# Autodesk Inventor assembly: PruebaIntegracion
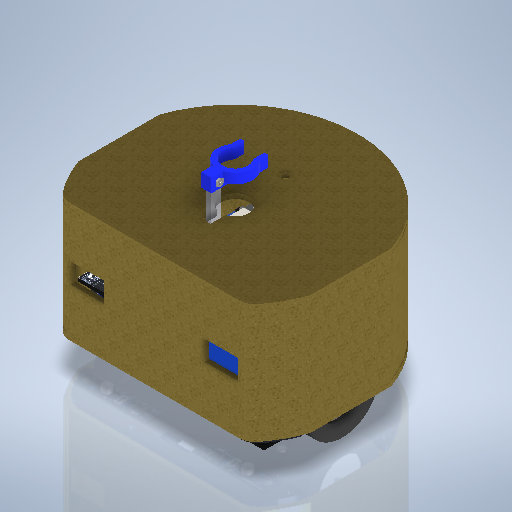
[picture p0: Inventor's stored thumbnail of the model, 512x512]
Saved by Autodesk Inventor 2025.2 (Build 292293000, 293)
## iProperties
Created: 2025-04-23
Part Number: PruebaIntegracion
Document SubType Name: Assembly
Designer: cdavi
Author: cdavi
## Documents named in this file (34)
- D:\Documentos\GIRoM\Atta-Bot-STEM\Chasis\Rediseño_Diego&Carlos\PruebaIntegracion.iam
- D:\Documentos\GIRoM\Atta-Bot-STEM\Chasis\Rediseño_Diego&Carlos\base_chasis_v5\base_chasis_v4-dimsAjustadas.ipt
- D:\Documentos\GIRoM\Atta-Bot-STEM\Chasis\Rediseño_Diego&Carlos\base_chasis_v5.ipt
- D:\Documentos\GIRoM\Atta-Bot-STEM\Chasis\Rediseño_Diego&Carlos\base_nivel2.ipt
- D:\Documentos\GIRoM\Atta-Bot-STEM\Chasis\Rediseño_Diego&Carlos\spacers\hexagonal_spacer_MF_M3_H20_HEX5.5_FTD6_MTL6.ipt
- D:\Documentos\GIRoM\Atta-Bot-STEM\Chasis\Rediseño_Diego&Carlos\spacers\hexagonal_spacer_MF_M3_H06_HEX5.5_FTD3_MTL6.ipt
- D:\Documentos\GIRoM\Atta-Bot-STEM\Chasis\Rediseño_Diego&Carlos\base_powerboost.ipt
- D:\Documentos\GIRoM\Atta-Bot-STEM\Chasis\Rediseño_Diego&Carlos\ideaboard.ipt
- D:\Documentos\GIRoM\Atta-Bot-STEM\Chasis\Rediseño_Diego&Carlos\sensorFrontal.ipt
- D:\Documentos\GIRoM\Atta-Bot-STEM\Chasis\Rediseño_Diego&Carlos\sensorInferior.ipt
- D:\Documentos\GIRoM\Atta-Bot-STEM\Chasis\Rediseño_Diego&Carlos\powerboost.ipt
- D:\Documentos\GIRoM\Atta-Bot-STEM\Chasis\Rediseño_Diego&Carlos\bateria.ipt
- D:\Documentos\GIRoM\Atta-Bot-STEM\Chasis\Rediseño_Diego&Carlos\soporteMotor.ipt
- D:\Documentos\GIRoM\Atta-Bot-STEM\Chasis\Rediseño_Diego&Carlos\motor.ipt
- D:\Documentos\GIRoM\Atta-Bot-STEM\Chasis\Rediseño_Diego&Carlos\llanta.ipt
- D:\Documentos\GIRoM\Atta-Bot-STEM\Chasis\Rediseño_Diego&Carlos\ball_caster.ipt
- D:\Documentos\GIRoM\Atta-Bot-STEM\Chasis\Rediseño_Diego&Carlos\switch.ipt
- D:\Documentos\GIRoM\Atta-Bot-STEM\Chasis\Rediseño_Diego&Carlos\Tower Pro MG90S Micro servo.ipt
- D:\Documentos\GIRoM\Atta-Bot-STEM\Chasis\Rediseño_Diego&Carlos\EngraneMod_v2.ipt
- D:\Documentos\GIRoM\Atta-Bot-STEM\Chasis\Rediseño_Diego&Carlos\sujetador_cremallera.ipt
- D:\Documentos\GIRoM\Atta-Bot-STEM\Chasis\Rediseño_Diego&Carlos\cremallera_v2\cremallera-01.ipt
- D:\Documentos\GIRoM\Atta-Bot-STEM\Chasis\Rediseño_Diego&Carlos\cremallera_v2.ipt
- D:\Documentos\GIRoM\Atta-Bot-STEM\Chasis\Rediseño_Diego&Carlos\sujetador_marcador_v2.ipt
- D:\Documentos\GIRoM\Atta-Bot-STEM\Chasis\Rediseño_Diego&Carlos\SoporteServo.ipt
- D:\Documentos\GIRoM\Atta-Bot-STEM\Chasis\Rediseño_Diego&Carlos\spacers\hexagonal_spacer_MF_M3_H08_HEX5_FTD4_MTL8.ipt
- D:\Documentos\GIRoM\Atta-Bot-STEM\Chasis\Rediseño_Diego&Carlos\Content Center Files\en-US\ISO 4032(2)\ISO 4032 - M3 - ISO.ipt
- D:\Documentos\GIRoM\Atta-Bot-STEM\Chasis\Rediseño_Diego&Carlos\Content Center Files\en-US\ISO 7045  Z\ISO 7045 - M3 x 6_ - 4.8 - Z - ISO.ipt
- D:\Documentos\GIRoM\Atta-Bot-STEM\Chasis\Rediseño_Diego&Carlos\Content Center Files\en-US\ISO 4762(2)\ISO 4762 - M3 x 12ISO.ipt
- D:\Documentos\GIRoM\Atta-Bot-STEM\Chasis\Rediseño_Diego&Carlos\Content Center Files\en-US\ISO 4032(2)\ISO 4032 - M2 - ISO.ipt
- D:\Documentos\GIRoM\Atta-Bot-STEM\Chasis\Rediseño_Diego&Carlos\Content Center Files\en-US\ISO 4762(2)\ISO 4762 - M2 x 8ISO.ipt
- D:\Documentos\GIRoM\Atta-Bot-STEM\Chasis\Rediseño_Diego&Carlos\Content Center Files\en-US\ISO 4762(2)\ISO 4762 - M2 x 12ISO.ipt
- D:\Documentos\GIRoM\Atta-Bot-STEM\Chasis\Rediseño_Diego&Carlos\Content Center Files\en-US\ISO 7045  Z\ISO 7045 - M1,6 x 6_ - 4.8 - Z - ISO.ipt
- D:\Documentos\GIRoM\Atta-Bot-STEM\Chasis\Rediseño_Diego&Carlos\Content Center Files\en-US\ISO 4762(2)\ISO 4762 - M3 x 8ISO.ipt
- D:\Documentos\GIRoM\Diseño mecánico\carcasa.ipt
## Components (106 placed, 31 different names)
1. carcasa:1 — Mate:217, Mate:218, Mate:219
2. hexagonal_spacer_MF_M3_H20_HEX5.5_FTD6_MTL6:1 — Mate:3, Mate:4, Mate:210, Mate:214
3. hexagonal_spacer_MF_M3_H20_HEX5.5_FTD6_MTL6:2 — Mate:5, Mate:6, Mate:211, Mate:212, Mate:216
4. hexagonal_spacer_MF_M3_H20_HEX5.5_FTD6_MTL6:3 — Mate:7, Mate:8, Mate:215
5. hexagonal_spacer_MF_M3_H20_HEX5.5_FTD6_MTL6:4 — Mate:9, Mate:10, Mate:213
6. hexagonal_spacer_MF_M3_H08_HEX5_FTD4_MTL8:2
7. hexagonal_spacer_MF_M3_H08_HEX5_FTD4_MTL8:1
8. hexagonal_spacer_MF_M3_H08_HEX5_FTD4_MTL8:3
9. hexagonal_spacer_MF_M3_H08_HEX5_FTD4_MTL8:4
10. hexagonal_spacer_MF_M3_H06_HEX5.5_FTD3_MTL6:2 — Mate:44, Mate:45
11. hexagonal_spacer_MF_M3_H06_HEX5.5_FTD3_MTL6:3 — Mate:48, Mate:49
12. hexagonal_spacer_MF_M3_H06_HEX5.5_FTD3_MTL6:1 — Mate:42, Mate:43, Mate:50, Mate:51
13. hexagonal_spacer_MF_M3_H06_HEX5.5_FTD3_MTL6:4 — Mate:46, Mate:47, Mate:52
14. hexagonal_spacer_MF_M3_H06_HEX5.5_FTD3_MTL6:5 — Mate:53, Mate:54, Mate:68, Mate:69, Mate:70
15. hexagonal_spacer_MF_M3_H06_HEX5.5_FTD3_MTL6:6 — Mate:55, Mate:56, Mate:66, Mate:67, Mate:73
16. ISO 4032 M3:37 — Mate:199, Mate:83
17. ISO 4032 M3:38 — Mate:201, Mate:85
18. ISO 7045 Z M3 x 6 - 4.8 - Z:25 — Insert:14
19. ISO 7045 Z M3 x 6 - 4.8 - Z:26 — Insert:15
20. ISO 4032 M3:39 — Insert:16
21. ISO 4032 M3:40 — Insert:17
22. ISO 4032 M3:41 — Insert:18
23. ISO 4032 M3:42 — Insert:19
24. ISO 4032 M3:43 — Insert:5
25. ISO 4032 M3:44 — Insert:6
26. ISO 4032 M3:45 — Insert:7
27. ISO 4032 M3:46 — Insert:8
28. ISO 7045 Z M3 x 6 - 4.8 - Z:27 — Insert:9
29. ISO 7045 Z M3 x 6 - 4.8 - Z:28 — Insert:10
30. ISO 4762 M3 x 12:5 — Insert:114
31. ISO 4762 M3 x 12:6 — Mate:115, Mate:116
32. ISO 7045 Z M3 x 6 - 4.8 - Z:29 — Mate:89, Mate:90
33. ISO 7045 Z M3 x 6 - 4.8 - Z:30 — Mate:91, Mate:92
34. ISO 7045 Z M3 x 6 - 4.8 - Z:31 — Mate:93, Mate:94
35. ISO 7045 Z M3 x 6 - 4.8 - Z:32 — Mate:95, Mate:96
36. ISO 4032 M3:47 — Mate:58, Mate:215
37. ISO 4032 M3:48 — Mate:60, Mate:216
38. ISO 4032 M3:49 — Mate:63, Mate:214
39. ISO 4032 M3:50 — Mate:64, Mate:213
40. ISO 4032 M3:51 — Mate:70, Mate:71
41. ISO 4032 M3:52 — Mate:72, Mate:73
42. ISO 7045 Z M3 x 6 - 4.8 - Z:33 — Mate:74, Mate:75
43. ISO 7045 Z M3 x 6 - 4.8 - Z:34 — Mate:76, Mate:77
44. ISO 7045 Z M3 x 6 - 4.8 - Z:35 — Mate:78, Mate:79
45. ISO 7045 Z M3 x 6 - 4.8 - Z:36 — Mate:80, Mate:81
46. ISO 4032 M2:18 — Mate:189, Mate:190
47. ISO 4032 M2:19 — Mate:191, Mate:192
48. ISO 4032 M2:20 — Mate:194, Mate:197
49. ISO 4032 M2:21 — Mate:196
50. ISO 4762 M2 x 8:19 — Mate:148, Mate:149, Mate:154
51. ISO 4762 M2 x 8:20 — Mate:150, Mate:151, Mate:152
52. ISO 4032 M2:22 — Mate:152, Mate:153
53. ISO 4032 M2:23 — Mate:154, Mate:155
54. ISO 4032 M2:24 — Mate:160, Mate:161
55. ISO 4032 M2:25 — Mate:162, Mate:163
56. ISO 4032 M2:26 — Mate:164, Mate:165
57. ISO 4032 M2:27 — Mate:166, Mate:167
58. ISO 4762 M2 x 8:21 — Mate:160
59. ISO 4762 M2 x 8:22 — Mate:162
60. ISO 4762 M2 x 8:23 — Mate:166
61. ISO 4762 M2 x 8:24 — Mate:164
62. ISO 4762 M2 x 8:25 — Mate:97, Mate:98, Mate:110, Mate:191
63. ISO 4762 M2 x 8:26 — Mate:99, Mate:100, Mate:112, Mate:189
64. ISO 4762 M2 x 12:7
65. ISO 4762 M2 x 12:8
66. ISO 4032 M2:28 — Mate:106
67. ISO 4032 M2:29 — Mate:107
68. ISO 4032 M2:30 — Mate:109, Mate:110
69. ISO 4032 M2:31 — Mate:111, Mate:112
70. ISO 7045 Z M1,6 x 6 - 4.8 - Z:4 — Mate:156, Mate:157
71. ISO 7045 Z M1,6 x 6 - 4.8 - Z:5 — Mate:158, Mate:159
72. bateria:1 — Mate:119, Mate:120
73. soporteMotor:1 — Mate:117, Mate:118, Angle:8, Mate:124, Tangent:2
74. soporteMotor:2 — Mate:119, Mate:122, Tangent:1, Mate:181, Angle:12, Mate:182
75. motor:1 — Mate:122, Tangent:1, Mate:123, Mate:126, Flush:5, Mate:127
76. motor:2 — Mate:124, Tangent:2, Mate:125, Mate:128, Mate:129, Flush:6
77. llanta:1 — Mate:126, Flush:5, Mate:127
78. llanta:2 — Mate:128, Mate:129, Flush:6
79. ball_caster:1 — Tangent:3, Tangent:7, Mate:130, Mate:156, Mate:158
80. switch:1 — Mate:131, Mate:132, Mate:133, Mate:148, Mate:149, Mate:150, Mate:151
81. sensorInferior:2 — Angle:7, Mate:85, Insert:114, Mate:82
82. sensorInferior:1 — Angle:6, Mate:83, Mate:115, Mate:116, Mate:84
83. powerboost:1 — Mate:86, Mate:87, Mate:88, Mate:97, Mate:98, Mate:99, Mate:100, Mate:197
84. base_chasis_v4-dimsAjustadas:1 — Mate:1, Flush:8, Flush:4, Mate:3, Mate:4, Mate:5, Mate:6, Mate:7, Mate:8, Mate:9, Mate:10, Mate:82, Angle:6, Mate:84, Angle:7, Mate:117, Mate:118, Angle:8, Mate:120, Mate:123, Mate:125, Tangent:3, Tangent:7, Mate:130, Mate:131, Mate:132, Mate:133, Mate:153, Mate:155, Mate:157, Mate:159, Mate:161, Mate:163, Mate:165, Mate:167, Insert:5, Insert:6, Insert:7, Insert:8, Insert:9, Insert:10, Mate:181, Angle:12, Mate:182, Mate:199, Mate:201, Mate:217, Mate:218, Mate:219
85. base_powerboost:1 — Mate:86, Mate:87, Mate:88, Mate:89, Mate:90, Mate:91, Mate:92, Mate:93, Mate:94, Mate:95, Mate:96, Mate:106, Mate:107, Mate:109, Mate:111, Mate:190, Mate:192, Mate:194, Mate:196
86. SoporteServo:2 — Mate:186, Mate:187, Mate:188, Mate:209
87. base_nivel2:1 — Mate:42, Mate:43, Mate:44, Mate:45, Mate:46, Mate:47, Mate:48, Mate:49, Mate:53, Mate:54, Mate:55, Mate:56, Mate:58, Mate:60, Mate:63, Mate:64, Angle:4, Angle:5, Angle:9, Insert:14, Insert:15, Insert:16, Insert:17, Insert:18, Insert:19, Flush:7, Mate:186, Mate:187, Mate:210, Mate:211, Mate:212
88. SoporteServo:1 — Mate:208
89. ideaboard:1 — Mate:50, Mate:51, Mate:52, Mate:74, Mate:75, Mate:76, Mate:77, Mate:78, Mate:79, Mate:80, Mate:81
90. sensorFrontal:1 — Mate:66, Mate:67, Angle:4, Mate:72
91. sensorFrontal:2 — Mate:68, Mate:69, Angle:5, Mate:71
92. ISO 4032 M2:32 — Mate:208
93. ISO 4032 M2:33 — Mate:209
94. ISO 4762 M2 x 12:9
95. ISO 4762 M3 x 8:3 — Mate:202, Mate:203, Mate:206
96. ISO 4762 M3 x 8:4 — Mate:204, Mate:205, Mate:207
97. ISO 4032 M3:53 — Mate:169, Mate:206
98. ISO 4032 M3:54 — Mate:171, Mate:207
99. ISO 4762 M2 x 12:10
100. Tower Pro MG90S Micro servo:1 — Angle:9, Mate:136, Mate:138, Angle:10, Mate:143, Flush:7, Mate:188
101. EngraneMod_v2:1 — Mate:136, Mate:139, Mate:143
102. sujetador_cremallera:1 — Mate:138, Angle:10, Mate:139, Tangent:5, Tangent:6, Mate:140, Mate:203, Mate:205, Mate:169, Mate:171
103. cremallera-01:1 — Tangent:5, Tangent:6, Mate:140, Mate:141, Angle:11, Mate:142, Mate:202, Mate:204
104. sujetador_marcador_v2:1 — Mate:141, Angle:11, Mate:142, Mate:144, Mate:145, Mate:147
105. ISO 4762 M2 x 8:27 — Mate:144, Mate:145, Mate:146
106. ISO 4032 M2:34 — Mate:146, Mate:147
## Relationships (218: Mate 180, Insert 18, Angle 9, Tangent 6, Flush 5)
- Mate:1: base_chasis_v4-dimsAjustadas:1
- Flush:8: base_chasis_v4-dimsAjustadas:1
- Flush:4: base_chasis_v4-dimsAjustadas:1
- Mate:3: hexagonal_spacer_MF_M3_H20_HEX5.5_FTD6_MTL6:1 ↔ base_chasis_v4-dimsAjustadas:1
- Mate:4: hexagonal_spacer_MF_M3_H20_HEX5.5_FTD6_MTL6:1 ↔ base_chasis_v4-dimsAjustadas:1
- Mate:5: hexagonal_spacer_MF_M3_H20_HEX5.5_FTD6_MTL6:2 ↔ base_chasis_v4-dimsAjustadas:1
- Mate:6: hexagonal_spacer_MF_M3_H20_HEX5.5_FTD6_MTL6:2 ↔ base_chasis_v4-dimsAjustadas:1
- Mate:7: hexagonal_spacer_MF_M3_H20_HEX5.5_FTD6_MTL6:3 ↔ base_chasis_v4-dimsAjustadas:1
- Mate:8: hexagonal_spacer_MF_M3_H20_HEX5.5_FTD6_MTL6:3 ↔ base_chasis_v4-dimsAjustadas:1
- Mate:9: hexagonal_spacer_MF_M3_H20_HEX5.5_FTD6_MTL6:4 ↔ base_chasis_v4-dimsAjustadas:1
- Mate:10: hexagonal_spacer_MF_M3_H20_HEX5.5_FTD6_MTL6:4 ↔ base_chasis_v4-dimsAjustadas:1
- [Mate]: hexagonal_spacer_MF_M3_H08_HEX5_FTD4_MTL8:2 ↔ base_chasis_v4-dimsAjustadas:1
- [Mate]: hexagonal_spacer_MF_M3_H08_HEX5_FTD4_MTL8:2 ↔ base_chasis_v4-dimsAjustadas:1
- [Mate]: hexagonal_spacer_MF_M3_H08_HEX5_FTD4_MTL8:1 ↔ base_chasis_v4-dimsAjustadas:1
- [Mate]: hexagonal_spacer_MF_M3_H08_HEX5_FTD4_MTL8:1 ↔ base_chasis_v4-dimsAjustadas:1
- [Mate]: hexagonal_spacer_MF_M3_H08_HEX5_FTD4_MTL8:3 ↔ base_chasis_v4-dimsAjustadas:1
- [Mate]: hexagonal_spacer_MF_M3_H08_HEX5_FTD4_MTL8:3 ↔ base_chasis_v4-dimsAjustadas:1
- [Mate]: hexagonal_spacer_MF_M3_H08_HEX5_FTD4_MTL8:4 ↔ base_chasis_v4-dimsAjustadas:1
- [Mate]: hexagonal_spacer_MF_M3_H08_HEX5_FTD4_MTL8:4 ↔ base_chasis_v4-dimsAjustadas:1
- [Mate]: hexagonal_spacer_MF_M3_H08_HEX5_FTD4_MTL8:3 ↔ base_powerboost:1
- [Mate]: hexagonal_spacer_MF_M3_H08_HEX5_FTD4_MTL8:2 ↔ base_powerboost:1
- [Mate]: hexagonal_spacer_MF_M3_H08_HEX5_FTD4_MTL8:2 ↔ base_powerboost:1
- [Mate]: base_nivel2:1 ↔ SoporteServo:1
- [Mate]: base_nivel2:1 ↔ SoporteServo:1
- [Mate]: base_nivel2:1 ↔ SoporteServo:1
- Mate:42: hexagonal_spacer_MF_M3_H06_HEX5.5_FTD3_MTL6:1 ↔ base_nivel2:1
- Mate:43: hexagonal_spacer_MF_M3_H06_HEX5.5_FTD3_MTL6:1 ↔ base_nivel2:1
- Mate:44: hexagonal_spacer_MF_M3_H06_HEX5.5_FTD3_MTL6:2 ↔ base_nivel2:1
- Mate:45: hexagonal_spacer_MF_M3_H06_HEX5.5_FTD3_MTL6:2 ↔ base_nivel2:1
- Mate:46: hexagonal_spacer_MF_M3_H06_HEX5.5_FTD3_MTL6:4 ↔ base_nivel2:1
- Mate:47: hexagonal_spacer_MF_M3_H06_HEX5.5_FTD3_MTL6:4 ↔ base_nivel2:1
- Mate:48: hexagonal_spacer_MF_M3_H06_HEX5.5_FTD3_MTL6:3 ↔ base_nivel2:1
- Mate:49: hexagonal_spacer_MF_M3_H06_HEX5.5_FTD3_MTL6:3 ↔ base_nivel2:1
- Mate:50: hexagonal_spacer_MF_M3_H06_HEX5.5_FTD3_MTL6:1 ↔ ideaboard:1
- Mate:51: hexagonal_spacer_MF_M3_H06_HEX5.5_FTD3_MTL6:1 ↔ ideaboard:1
- Mate:52: hexagonal_spacer_MF_M3_H06_HEX5.5_FTD3_MTL6:4 ↔ ideaboard:1
- Mate:53: hexagonal_spacer_MF_M3_H06_HEX5.5_FTD3_MTL6:5 ↔ base_nivel2:1
- Mate:54: hexagonal_spacer_MF_M3_H06_HEX5.5_FTD3_MTL6:5 ↔ base_nivel2:1
- Mate:55: hexagonal_spacer_MF_M3_H06_HEX5.5_FTD3_MTL6:6 ↔ base_nivel2:1
- Mate:56: hexagonal_spacer_MF_M3_H06_HEX5.5_FTD3_MTL6:6 ↔ base_nivel2:1
- Mate:58: ISO 4032 M3:47 ↔ base_nivel2:1
- Mate:60: ISO 4032 M3:48 ↔ base_nivel2:1
- Mate:63: ISO 4032 M3:49 ↔ base_nivel2:1
- Mate:64: ISO 4032 M3:50 ↔ base_nivel2:1
- Mate:66: hexagonal_spacer_MF_M3_H06_HEX5.5_FTD3_MTL6:6 ↔ sensorFrontal:1
- Mate:67: hexagonal_spacer_MF_M3_H06_HEX5.5_FTD3_MTL6:6 ↔ sensorFrontal:1
- Angle:4 (180 deg): base_nivel2:1 ↔ sensorFrontal:1
- Mate:68: hexagonal_spacer_MF_M3_H06_HEX5.5_FTD3_MTL6:5 ↔ sensorFrontal:2
- Mate:69: hexagonal_spacer_MF_M3_H06_HEX5.5_FTD3_MTL6:5 ↔ sensorFrontal:2
- Angle:5 (0 deg): base_nivel2:1 ↔ sensorFrontal:2
- Mate:70: hexagonal_spacer_MF_M3_H06_HEX5.5_FTD3_MTL6:5 ↔ ISO 4032 M3:51
- Mate:71: ISO 4032 M3:51 ↔ sensorFrontal:2
- Mate:72: ISO 4032 M3:52 ↔ sensorFrontal:1
- Mate:73: hexagonal_spacer_MF_M3_H06_HEX5.5_FTD3_MTL6:6 ↔ ISO 4032 M3:52
- Mate:74: ISO 7045 Z M3 x 6 - 4.8 - Z:33 ↔ ideaboard:1
- Mate:75: ISO 7045 Z M3 x 6 - 4.8 - Z:33 ↔ ideaboard:1
- Mate:76: ISO 7045 Z M3 x 6 - 4.8 - Z:34 ↔ ideaboard:1
- Mate:77: ISO 7045 Z M3 x 6 - 4.8 - Z:34 ↔ ideaboard:1
- Mate:78: ISO 7045 Z M3 x 6 - 4.8 - Z:35 ↔ ideaboard:1
- Mate:79: ISO 7045 Z M3 x 6 - 4.8 - Z:35 ↔ ideaboard:1
- Mate:80: ISO 7045 Z M3 x 6 - 4.8 - Z:36 ↔ ideaboard:1
- Mate:81: ISO 7045 Z M3 x 6 - 4.8 - Z:36 ↔ ideaboard:1
- Mate:82: sensorInferior:2 ↔ base_chasis_v4-dimsAjustadas:1
- Angle:6 (0 deg): sensorInferior:1 ↔ base_chasis_v4-dimsAjustadas:1
- Mate:83: ISO 4032 M3:37 ↔ sensorInferior:1
- Mate:84: sensorInferior:1 ↔ base_chasis_v4-dimsAjustadas:1
- Angle:7 (0 deg): sensorInferior:2 ↔ base_chasis_v4-dimsAjustadas:1
- Mate:85: ISO 4032 M3:38 ↔ sensorInferior:2
- Mate:86: powerboost:1 ↔ base_powerboost:1
- Mate:87: powerboost:1 ↔ base_powerboost:1
- Mate:88 (1 mm): powerboost:1 ↔ base_powerboost:1
- Mate:89: ISO 7045 Z M3 x 6 - 4.8 - Z:29 ↔ base_powerboost:1
- Mate:90: ISO 7045 Z M3 x 6 - 4.8 - Z:29 ↔ base_powerboost:1
- Mate:91: ISO 7045 Z M3 x 6 - 4.8 - Z:30 ↔ base_powerboost:1
- Mate:92: ISO 7045 Z M3 x 6 - 4.8 - Z:30 ↔ base_powerboost:1
- Mate:93: ISO 7045 Z M3 x 6 - 4.8 - Z:31 ↔ base_powerboost:1
- Mate:94: ISO 7045 Z M3 x 6 - 4.8 - Z:31 ↔ base_powerboost:1
- Mate:95: ISO 7045 Z M3 x 6 - 4.8 - Z:32 ↔ base_powerboost:1
- Mate:96: ISO 7045 Z M3 x 6 - 4.8 - Z:32 ↔ base_powerboost:1
- Mate:97: ISO 4762 M2 x 8:25 ↔ powerboost:1
- Mate:98: ISO 4762 M2 x 8:25 ↔ powerboost:1
- Mate:99: ISO 4762 M2 x 8:26 ↔ powerboost:1
- Mate:100: ISO 4762 M2 x 8:26 ↔ powerboost:1
- [Mate]: ISO 4762 M2 x 12:7 ↔ powerboost:1
- [Mate]: ISO 4762 M2 x 12:7 ↔ powerboost:1
- [Mate]: ISO 4762 M2 x 12:8 ↔ powerboost:1
- [Mate]: ISO 4762 M2 x 12:8 ↔ powerboost:1
- [Mate]: ISO 4762 M2 x 12:7 ↔ ISO 4032 M2:28
- Mate:106: ISO 4032 M2:28 ↔ base_powerboost:1
- Mate:107: ISO 4032 M2:29 ↔ base_powerboost:1
- [Mate]: ISO 4762 M2 x 12:8 ↔ ISO 4032 M2:29
- Mate:109: ISO 4032 M2:30 ↔ base_powerboost:1
- Mate:110: ISO 4762 M2 x 8:25 ↔ ISO 4032 M2:30
- Mate:111: ISO 4032 M2:31 ↔ base_powerboost:1
- Mate:112: ISO 4762 M2 x 8:26 ↔ ISO 4032 M2:31
- Insert:114: ISO 4762 M3 x 12:5 ↔ sensorInferior:2
- Mate:115: ISO 4762 M3 x 12:6 ↔ sensorInferior:1
- Mate:116: ISO 4762 M3 x 12:6 ↔ sensorInferior:1
- Mate:117: soporteMotor:1 ↔ base_chasis_v4-dimsAjustadas:1
- Mate:118: soporteMotor:1 ↔ base_chasis_v4-dimsAjustadas:1
- Angle:8 (0 deg): soporteMotor:1 ↔ base_chasis_v4-dimsAjustadas:1
- Mate:119: bateria:1 ↔ soporteMotor:2
- Mate:120: bateria:1 ↔ base_chasis_v4-dimsAjustadas:1
- [Mate] (1 mm): hexagonal_spacer_MF_M3_H08_HEX5_FTD4_MTL8:1 ↔ bateria:1
- Mate:122: soporteMotor:2 ↔ motor:1
- Tangent:1: soporteMotor:2 ↔ motor:1
- Mate:123: motor:1 ↔ base_chasis_v4-dimsAjustadas:1
- Mate:124: soporteMotor:1 ↔ motor:2
- Tangent:2: soporteMotor:1 ↔ motor:2
- Mate:125: motor:2 ↔ base_chasis_v4-dimsAjustadas:1
- Mate:126: motor:1 ↔ llanta:1
- Flush:5 (-3 mm): motor:1 ↔ llanta:1
- Mate:127: motor:1 ↔ llanta:1
- Mate:128: motor:2 ↔ llanta:2
- Mate:129: motor:2 ↔ llanta:2
- Flush:6 (-3 mm): motor:2 ↔ llanta:2
- Tangent:3: ball_caster:1 ↔ base_chasis_v4-dimsAjustadas:1
- Tangent:7: ball_caster:1 ↔ base_chasis_v4-dimsAjustadas:1
- Mate:130: ball_caster:1 ↔ base_chasis_v4-dimsAjustadas:1
- Mate:131: switch:1 ↔ base_chasis_v4-dimsAjustadas:1
- Mate:132: switch:1 ↔ base_chasis_v4-dimsAjustadas:1
- Mate:133 (0.2 mm): switch:1 ↔ base_chasis_v4-dimsAjustadas:1
- [Mate]: SoporteServo:1 ↔ Tower Pro MG90S Micro servo:1
- Angle:9 (180 deg): base_nivel2:1 ↔ Tower Pro MG90S Micro servo:1
- Mate:136: Tower Pro MG90S Micro servo:1 ↔ EngraneMod_v2:1
- Mate:138: Tower Pro MG90S Micro servo:1 ↔ sujetador_cremallera:1
- Angle:10 (0 deg): Tower Pro MG90S Micro servo:1 ↔ sujetador_cremallera:1
- Mate:139: EngraneMod_v2:1 ↔ sujetador_cremallera:1
- Tangent:5: sujetador_cremallera:1 ↔ cremallera-01:1
- Tangent:6: sujetador_cremallera:1 ↔ cremallera-01:1
- Mate:140: sujetador_cremallera:1 ↔ cremallera-01:1
- Mate:141: cremallera-01:1 ↔ sujetador_marcador_v2:1
- Angle:11 (0 deg): cremallera-01:1 ↔ sujetador_marcador_v2:1
- Mate:142: cremallera-01:1 ↔ sujetador_marcador_v2:1
- Mate:143: Tower Pro MG90S Micro servo:1 ↔ EngraneMod_v2:1
- Mate:144: sujetador_marcador_v2:1 ↔ ISO 4762 M2 x 8:27
- Mate:145: sujetador_marcador_v2:1 ↔ ISO 4762 M2 x 8:27
- Mate:146: ISO 4762 M2 x 8:27 ↔ ISO 4032 M2:34
- Mate:147: sujetador_marcador_v2:1 ↔ ISO 4032 M2:34
- Mate:148: ISO 4762 M2 x 8:19 ↔ switch:1
- Mate:149: ISO 4762 M2 x 8:19 ↔ switch:1
- Mate:150: ISO 4762 M2 x 8:20 ↔ switch:1
- Mate:151: ISO 4762 M2 x 8:20 ↔ switch:1
- Mate:152: ISO 4762 M2 x 8:20 ↔ ISO 4032 M2:22
- Mate:153: ISO 4032 M2:22 ↔ base_chasis_v4-dimsAjustadas:1
- Mate:154: ISO 4762 M2 x 8:19 ↔ ISO 4032 M2:23
- Mate:155: ISO 4032 M2:23 ↔ base_chasis_v4-dimsAjustadas:1
- Mate:156: ISO 7045 Z M1,6 x 6 - 4.8 - Z:4 ↔ ball_caster:1
- Mate:157: ISO 7045 Z M1,6 x 6 - 4.8 - Z:4 ↔ base_chasis_v4-dimsAjustadas:1
- Mate:158: ISO 7045 Z M1,6 x 6 - 4.8 - Z:5 ↔ ball_caster:1
- Mate:159: ISO 7045 Z M1,6 x 6 - 4.8 - Z:5 ↔ base_chasis_v4-dimsAjustadas:1
- [Insert]: ISO 4762 M2 x 8:21 ↔ soporteMotor:2
- [Insert]: ISO 4762 M2 x 8:22 ↔ soporteMotor:2
- [Insert]: ISO 4762 M2 x 8:23 ↔ soporteMotor:1
- [Insert]: ISO 4762 M2 x 8:24 ↔ soporteMotor:1
- Mate:160: ISO 4032 M2:24 ↔ ISO 4762 M2 x 8:21
- Mate:161: ISO 4032 M2:24 ↔ base_chasis_v4-dimsAjustadas:1
- Mate:162: ISO 4032 M2:25 ↔ ISO 4762 M2 x 8:22
- Mate:163: ISO 4032 M2:25 ↔ base_chasis_v4-dimsAjustadas:1
- Mate:164: ISO 4032 M2:26 ↔ ISO 4762 M2 x 8:24
- Mate:165: ISO 4032 M2:26 ↔ base_chasis_v4-dimsAjustadas:1
- Mate:166: ISO 4032 M2:27 ↔ ISO 4762 M2 x 8:23
- Mate:167: ISO 4032 M2:27 ↔ base_chasis_v4-dimsAjustadas:1
- Insert:5: ISO 4032 M3:43 ↔ base_chasis_v4-dimsAjustadas:1
- Insert:6: ISO 4032 M3:44 ↔ base_chasis_v4-dimsAjustadas:1
- Insert:7: ISO 4032 M3:45 ↔ base_chasis_v4-dimsAjustadas:1
- Insert:8: ISO 4032 M3:46 ↔ base_chasis_v4-dimsAjustadas:1
- Insert:9: ISO 7045 Z M3 x 6 - 4.8 - Z:27 ↔ base_chasis_v4-dimsAjustadas:1
- Insert:10: ISO 7045 Z M3 x 6 - 4.8 - Z:28 ↔ base_chasis_v4-dimsAjustadas:1
- Mate:169: ISO 4032 M3:53 ↔ sujetador_cremallera:1
- Mate:171: ISO 4032 M3:54 ↔ sujetador_cremallera:1
- [Mate]: ISO 4762 M2 x 12:10 ↔ Tower Pro MG90S Micro servo:1
- [Mate]: ISO 4762 M2 x 12:10 ↔ Tower Pro MG90S Micro servo:1
- [Insert]: ISO 4762 M2 x 12:9 ↔ Tower Pro MG90S Micro servo:1
- [Mate]: ISO 4032 M2:33 ↔ ISO 4762 M2 x 12:9
- [Mate]: ISO 4032 M2:32 ↔ ISO 4762 M2 x 12:10
- Insert:14: ISO 7045 Z M3 x 6 - 4.8 - Z:25 ↔ base_nivel2:1
- Insert:15: ISO 7045 Z M3 x 6 - 4.8 - Z:26 ↔ base_nivel2:1
- Insert:16: ISO 4032 M3:39 ↔ base_nivel2:1
- Insert:17: ISO 4032 M3:40 ↔ base_nivel2:1
- Insert:18: ISO 4032 M3:41 ↔ base_nivel2:1
- Insert:19: ISO 4032 M3:42 ↔ base_nivel2:1
- Flush:7: base_nivel2:1 ↔ Tower Pro MG90S Micro servo:1
- Mate:181: soporteMotor:2 ↔ base_chasis_v4-dimsAjustadas:1
- Angle:12 (0 deg): soporteMotor:2 ↔ base_chasis_v4-dimsAjustadas:1
- Mate:182: soporteMotor:2 ↔ base_chasis_v4-dimsAjustadas:1
- Mate:186: SoporteServo:2 ↔ base_nivel2:1
- Mate:187: SoporteServo:2 ↔ base_nivel2:1
- Mate:188: SoporteServo:2 ↔ Tower Pro MG90S Micro servo:1
- Mate:189: ISO 4032 M2:18 ↔ ISO 4762 M2 x 8:26
- Mate:190: ISO 4032 M2:18 ↔ base_powerboost:1
- Mate:191: ISO 4032 M2:19 ↔ ISO 4762 M2 x 8:25
- Mate:192: ISO 4032 M2:19 ↔ base_powerboost:1
- [Mate]: ISO 4032 M2:20 ↔ ISO 4762 M2 x 12:8
- Mate:194: ISO 4032 M2:20 ↔ base_powerboost:1
- [Mate]: ISO 4032 M2:21 ↔ ISO 4762 M2 x 12:7
- Mate:196: ISO 4032 M2:21 ↔ base_powerboost:1
- Mate:197: ISO 4032 M2:20 ↔ powerboost:1
- Mate:199: ISO 4032 M3:37 ↔ base_chasis_v4-dimsAjustadas:1
- Mate:201: ISO 4032 M3:38 ↔ base_chasis_v4-dimsAjustadas:1
- Mate:202: ISO 4762 M3 x 8:3 ↔ cremallera-01:1
- Mate:203: ISO 4762 M3 x 8:3 ↔ sujetador_cremallera:1
- Mate:204: ISO 4762 M3 x 8:4 ↔ cremallera-01:1
- Mate:205: ISO 4762 M3 x 8:4 ↔ sujetador_cremallera:1
- Mate:206: ISO 4762 M3 x 8:3 ↔ ISO 4032 M3:53
- Mate:207: ISO 4762 M3 x 8:4 ↔ ISO 4032 M3:54
- Mate:208: SoporteServo:1 ↔ ISO 4032 M2:32
- Mate:209: SoporteServo:2 ↔ ISO 4032 M2:33
- Mate:210: hexagonal_spacer_MF_M3_H20_HEX5.5_FTD6_MTL6:1 ↔ base_nivel2:1
- Mate:211: hexagonal_spacer_MF_M3_H20_HEX5.5_FTD6_MTL6:2 ↔ base_nivel2:1
- Mate:212: hexagonal_spacer_MF_M3_H20_HEX5.5_FTD6_MTL6:2 ↔ base_nivel2:1
- Mate:213: hexagonal_spacer_MF_M3_H20_HEX5.5_FTD6_MTL6:4 ↔ ISO 4032 M3:50
- Mate:214: hexagonal_spacer_MF_M3_H20_HEX5.5_FTD6_MTL6:1 ↔ ISO 4032 M3:49
- Mate:215: hexagonal_spacer_MF_M3_H20_HEX5.5_FTD6_MTL6:3 ↔ ISO 4032 M3:47
- Mate:216: hexagonal_spacer_MF_M3_H20_HEX5.5_FTD6_MTL6:2 ↔ ISO 4032 M3:48
- Mate:217: carcasa:1 ↔ base_chasis_v4-dimsAjustadas:1
- Mate:218: carcasa:1 ↔ base_chasis_v4-dimsAjustadas:1
- Mate:219: carcasa:1 ↔ base_chasis_v4-dimsAjustadas:1
## Named parameters: Finish10_Area = 2.70707, Finish11_Area = 34.5669, Finish12_Area = 34.5669, Finish13_Area = 34.5669, Finish14_Area = 241.215, Finish15_Area = 241.215, Finish16_Area = 0.56205, Finish17_Area = 0.56205, Finish18_Area = 1.1241, Finish19_Area = 1.1241, Finish1_Area = 453.766, Finish20_Area = 5.43503, Finish21_Area = 5.43503, Finish2_Area = 0.953201, Finish2_Thickness = 0.05 mm, Finish3_Area = 2.8596, Finish3_Thickness = 0.05 mm, Finish4_Area = 412.295, Finish5_Area = 41.4714, Finish6_Area = 2.70707, Finish7_Area = 13.3512, Finish8_Area = 13.3512, Finish9_Area = 2.70707
note: some values were not read from the file. Shown as the stored number, unit unknown: "Finish10_Area", "Finish11_Area", "Finish12_Area", "Finish13_Area", "Finish14_Area", "Finish15_Area", "Finish16_Area", "Finish17_Area", "Finish18_Area", "Finish19_Area", "Finish1_Area", "Finish20_Area", "Finish21_Area", "Finish2_Area", "Finish3_Area", "Finish4_Area", "Finish5_Area", "Finish6_Area", "Finish7_Area", "Finish8_Area", "Finish9_Area".
